# Autodesk Inventor assembly: Assembly146-01
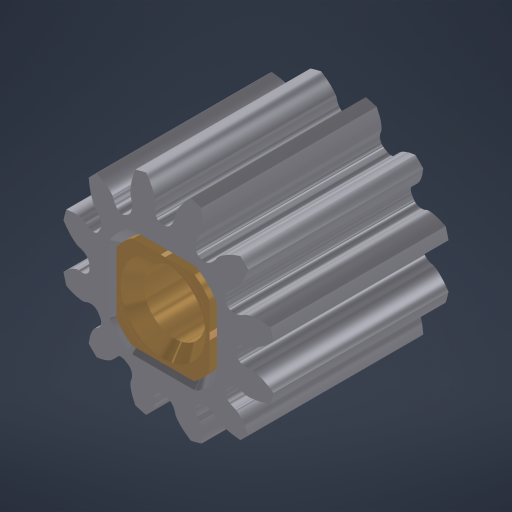
[picture p0: Inventor's stored thumbnail of the model, 512x512]
Saved by Autodesk Inventor 2023.2 (Build 272271000, 271)
## iProperties
Created: 2022-08-02
Part Number: Assembly146-01
Document SubType Name: Assembly
Designer: ylu12
Author: ylu12
## Documents named in this file (4)
- D:\CAD\Parts\standard\Motion\Gears\HS\HS Gear\HS 12T Gear, Circle.iam
- D:\CAD\Parts\standard\Motion\Adapters\HS Shaft Adapter Circle.ipt
- D:\CAD\Parts\standard\Motion\Gears\HS\Reference parts\HS 12T Gear, No Insert.ipt
- D:\CAD\Parts\standard\Motion\Gears\HS\HS Gear.iam
## Components (2 placed, 2 different names)
1. Circle — Mate:1, Mate:2, Flush:1
2. 12T — Mate:5, Mate:6, Flush:3
## Relationships (6: Mate 4, Flush 2)
- Mate:1: Circle
- Mate:2: Circle
- Flush:1 (6.35 mm): Circle
- Mate:5: 12T
- Mate:6: 12T
- Flush:3: 12T
